# Autodesk Inventor assembly: head_div
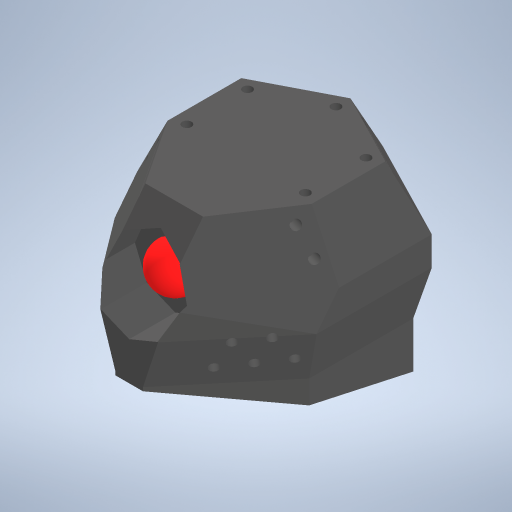
[picture p0: Inventor's stored thumbnail of the model, 512x512]
Saved by Autodesk Inventor 2024.1 (Build 281209000, 209)
## iProperties
Created: 2024-03-01
Part Number: head_div
Document SubType Name: Assembly
Designer: hibik
Author: hibik
## Documents named in this file (3)
- C:\Users\hibik\Desktop\ロボメカ\HR\2024.02.11 Rl\02.11 ProtType\head\head_div.iam
- C:\Users\hibik\Desktop\ロボメカ\HR\2024.02.11 Rl\02.11 ProtType\head\head_bace_div_under.ipt
- C:\Users\hibik\Desktop\ロボメカ\HR\2024.02.11 Rl\02.11 ProtType\head\head_bace_div_upper.ipt
## Components (2 placed, 2 different names)
1. head_bace_div_under:1 — メイト:1, フラッシュ:1, フラッシュ:2
2. head_bace_div_upper:1 — メイト:1, フラッシュ:1, フラッシュ:2
## Relationships (3: Flush 2, Mate 1)
- メイト:1 [Mate]: head_bace_div_under:1 ↔ head_bace_div_upper:1
- フラッシュ:1 [Flush]: head_bace_div_under:1 ↔ head_bace_div_upper:1
- フラッシュ:2 [Flush]: head_bace_div_under:1 ↔ head_bace_div_upper:1
